# Autodesk Inventor assembly: A Drive
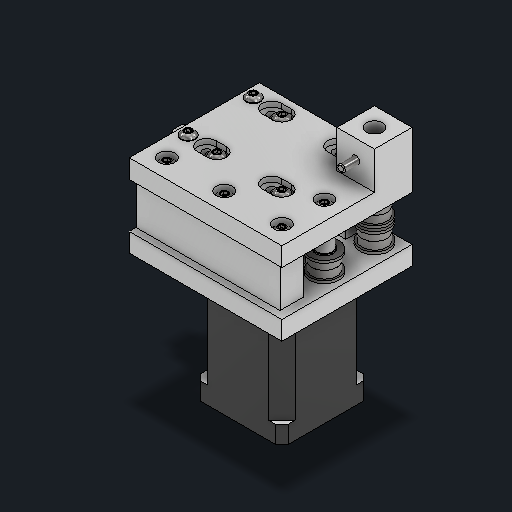
[picture p0: Inventor's stored thumbnail of the model, 512x512]
Saved by Autodesk Inventor 2025.1 (Build 291241020, 241B)
## iProperties
Created: 2025-05-09
Part Number: A Drive
Document SubType Name: Assembly
Designer: AdminForWorker
Title: A Drive
Author: AdminForWorker
## Documents named in this file (10)
- C:\Users\Joshua Eah\Documents\Voron 0.2\CAD\Master Assembly\Motion\AB Drives\Drives\A Drive.iam
- C:\Users\Joshua Eah\Documents\Voron 0.2\CAD\Machined Parts\AB Drives\A Drive\A Drive Assembly.iam
- C:\Users\Joshua Eah\Documents\Voron 0.2\CAD\Master Assembly\Hardware\M3x35 BHCS.ipt
- C:\Users\Joshua Eah\Documents\Voron 0.2\CAD\Master Assembly\Hardware\M3x30 BHCS.ipt
- C:\Users\Joshua Eah\Documents\Voron 0.2\CAD\Master Assembly\Hardware\M3x10 BHCS.ipt
- C:\Users\Joshua Eah\Documents\Voron 0.2\CAD\Master Assembly\Hardware\M3 Hexnut.ipt
- C:\Users\Joshua Eah\Documents\Voron 0.2\CAD\Master Assembly\Hardware\F623 Stack.iam
- C:\Users\Joshua Eah\Documents\Voron 0.2\CAD\Master Assembly\Hardware\M3_Washer.ipt
- C:\Users\Joshua Eah\Documents\Voron 0.2\CAD\Master Assembly\Motion\AB Drives\Motor Assembly\Nema14.ipt
- C:\Users\Joshua Eah\Documents\Voron 0.2\CAD\Master Assembly\Motion\AB Drives\Motor Assembly\GT2 20T 6mm Pulley.iam
## Components (26 placed, 9 different names)
1. A Drive Assembly:1 [sub-assembly] — Insert:3, Insert:5, Insert:7, Insert:8, Insert:9, Mate:4, Mate:9
2. Nema14:1 — Mate:5, Mate:6, Mate:7, Mate:8, Mate:9
3. GT2 20T 6mm Pulley:1 [sub-assembly] — Mate:6, Mate:7
4. M3x10 BHCS:1
5. M3x35 BHCS:1 — Mate:2, Mate:8
6. M3x35 BHCS:2 — Mate:1
7. M3x35 BHCS:3
8. M3x35 BHCS:4
9. M3x35 BHCS:5
10. M3x35 BHCS:6
11. M3x35 BHCS:7 — Insert:6, Mate:5
12. M3x35 BHCS:8 — Mate:3
13. M3x35 BHCS:9 — Insert:3, Insert:4
14. M3x30 BHCS:1
15. M3x30 BHCS:2 — Insert:5
16. M3 Hexnut:1
17. M3 Hexnut:2
18. M3 Hexnut:3
19. M3 Hexnut:4 — Insert:4
20. M3_Washer:1 — Mate:3, Mate:4
21. M3_Washer:2 — Insert:6, Insert:7
22. M3_Washer:3 — Mate:2, Insert:9
23. M3_Washer:4 — Mate:1, Insert:8
24. F623 Stack:1 [sub-assembly]
25. F623 Stack:2 [sub-assembly]
26. F623 Stack:3 [sub-assembly]
## Relationships (18: Insert 9, Mate 9)
- [Insert]: A Drive Assembly:1 ↔ M3x10 BHCS:1
- [Insert]: A Drive Assembly:1 ↔ M3x35 BHCS:4
- Insert:3: A Drive Assembly:1 ↔ M3x35 BHCS:9
- Insert:4: M3x35 BHCS:9 ↔ M3 Hexnut:4
- Insert:5: A Drive Assembly:1 ↔ M3x30 BHCS:2
- Insert:6: M3x35 BHCS:7 ↔ M3_Washer:2
- Insert:7: A Drive Assembly:1 ↔ M3_Washer:2
- Mate:1: M3x35 BHCS:2 ↔ M3_Washer:4
- Mate:2: M3x35 BHCS:1 ↔ M3_Washer:3
- Mate:3: M3x35 BHCS:8 ↔ M3_Washer:1
- Insert:8: A Drive Assembly:1 ↔ M3_Washer:4
- Insert:9: A Drive Assembly:1 ↔ M3_Washer:3
- Mate:4: A Drive Assembly:1 ↔ M3_Washer:1
- Mate:5: Nema14:1 ↔ M3x35 BHCS:7
- Mate:6: Nema14:1 ↔ GT2 20T 6mm Pulley:1
- Mate:7 (5.35 mm): Nema14:1 ↔ GT2 20T 6mm Pulley:1
- Mate:8: Nema14:1 ↔ M3x35 BHCS:1
- Mate:9: A Drive Assembly:1 ↔ Nema14:1
